# Autodesk Inventor assembly: 537245 FNC-12
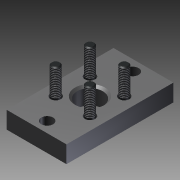
[picture p0: Inventor's stored thumbnail of the model, 180x180]
Saved by Autodesk Inventor 2011 SP1 (Build 150282100, 282)
## iProperties
Created: 2018-05-28
Part Number: 537245 FNC-12
Catalog Web Link: www.cadenas.de
Description: FNC-Flange mounting
Vendor: FESTO
Document SubType Name: Assembly
Designer: psAdmin
Manufacturer: FESTO
Mass: 79 g
Category: PARTsolutions
Company: FESTO
Title: 537245 FNC-12
Author: Cadenas PARTsolutions
Comments: Flange mounting
PSOL_IDENT_0: {$CADENAS_DATA\23d-libs\festo\parts\f\fnc\fnc_asmtab.prj},179 {VTYP=3D},{STYP=ASSTAB},{NB=537245 FNC
PSOL_IDENT_1: -12},{LINA=537245 FNC-12},{NN=FNC},{DATE=02.09.2015 15:05:29},{GEOMDATE=02.09.2015 15:05:29},{VERSIO
PSOL_IDENT_2: N=},{LINEID=80},{LINESUBID=-1},{WBVAR=}  {NB=537245 FNC-12},{LINA=537245 FNC-12},{KT=DUMMY},{TNR=537
PSOL_IDENT_3: 245},{TYP=FNC-12},{VERS=1},{D1=12.000},{D2=4.800},{D3=8.000},{E=28.000},{F=1.000},{FB=5.500},{MF=8.0
PSOL_IDENT_4: 00},{R=0.000},{T=3.000},{TF=40.000},{TG1=16.000},{UF=50.000},{CNSMASSEXACT=0.079},{ZZ=0},{DK=12},{D6
PSOL_IDENT_5: 912D=4.000},{D6912L=16.000},{PPATH=assemblies/fnc_asmtpl.prj}
NN: FNC
NT: Flange mounting
NB: 537245 FNC-12
NBSYN: $TNR. $TYP.
LINA: 537245 FNC-12
TNR: 537245
TYP: FNC-12
D1: 12.000
D2: 4.800
D3: 8.000
E: 28.000
F: 1.000
FB: 5.500
MF: 8.000
R: 0.000
T: 3.000
TF: 40.000
TG1: 16.000
UF: 50.000
CNSMASSEXACT: 0.079
SUPPLIER: FESTO
ARTICLENO: 537245 FNC-12
BOMINFO: 537245 FNC-12
CREATOR: CADENAS GmbH
## Documents named in this file (3)
- p:\temp\worker_3\2348_1500\cad_40_02018052900041801315782192d056f_000000_00_00_000001\537245 FNC-12.iam
- p:\temp\worker_3\2348_1500\cad_40_02018052900041801315782192d056f_000000_00_00_000001\537245 FNC-12---(F).ipt
- p:\temp\worker_3\2348_1500\cad_40_02018052900041801315782192d056f_000000_00_00_000001\DIN-6912 - M4x16(F).ipt
## Components (5 placed, 2 different names)
1. 537245 FNC-12---(F):1 — FNC_Schraube_1_XY@1 <-> MONTAGE_XY@2, FNC_Schraube_1_Z@1 <-> MONTAGE_Z@2, FNC_Schraube_2_XY@1 <-> MONTAGE_XY@3, FNC_Schraube_2_Z@1 <-> MONTAGE_Z@3, FNC_Schraube_2_YZ@1 <-> MONTAGE_YZ@3, FNC_Schraube_3_XY@1 <-> MONTAGE_XY@4, FNC_Schraube_3_Z@1 <-> MONTAGE_Z@4, FNC_Schraube_3_YZ@1 <-> MONTAGE_YZ@4, FNC_Schraube_4_XY@1 <-> MONTAGE_XY@5, FNC_Schraube_4_Z@1 <-> MONTAGE_Z@5
2. DIN-6912 - M4x16(F):1 — FNC_Schraube_1_XY@1 <-> MONTAGE_XY@2, FNC_Schraube_1_Z@1 <-> MONTAGE_Z@2
3. DIN-6912 - M4x16(F):2 — FNC_Schraube_2_XY@1 <-> MONTAGE_XY@3, FNC_Schraube_2_Z@1 <-> MONTAGE_Z@3, FNC_Schraube_2_YZ@1 <-> MONTAGE_YZ@3
4. DIN-6912 - M4x16(F):3 — FNC_Schraube_3_XY@1 <-> MONTAGE_XY@4, FNC_Schraube_3_Z@1 <-> MONTAGE_Z@4, FNC_Schraube_3_YZ@1 <-> MONTAGE_YZ@4
5. DIN-6912 - M4x16(F):4 — FNC_Schraube_4_XY@1 <-> MONTAGE_XY@5, FNC_Schraube_4_Z@1 <-> MONTAGE_Z@5
## Relationships (10: Flush 4, Mate 4, Angle 2)
- FNC_Schraube_1_XY@1 <-> MONTAGE_XY@2 [Flush]: 537245 FNC-12---(F):1 ↔ DIN-6912 - M4x16(F):1
- FNC_Schraube_1_Z@1 <-> MONTAGE_Z@2 [Mate]: 537245 FNC-12---(F):1 ↔ DIN-6912 - M4x16(F):1
- FNC_Schraube_2_XY@1 <-> MONTAGE_XY@3 [Flush]: 537245 FNC-12---(F):1 ↔ DIN-6912 - M4x16(F):2
- FNC_Schraube_2_Z@1 <-> MONTAGE_Z@3 [Mate]: 537245 FNC-12---(F):1 ↔ DIN-6912 - M4x16(F):2
- FNC_Schraube_2_YZ@1 <-> MONTAGE_YZ@3 [Angle] (0 deg): 537245 FNC-12---(F):1 ↔ DIN-6912 - M4x16(F):2
- FNC_Schraube_3_XY@1 <-> MONTAGE_XY@4 [Flush]: 537245 FNC-12---(F):1 ↔ DIN-6912 - M4x16(F):3
- FNC_Schraube_3_Z@1 <-> MONTAGE_Z@4 [Mate]: 537245 FNC-12---(F):1 ↔ DIN-6912 - M4x16(F):3
- FNC_Schraube_3_YZ@1 <-> MONTAGE_YZ@4 [Angle] (0 deg): 537245 FNC-12---(F):1 ↔ DIN-6912 - M4x16(F):3
- FNC_Schraube_4_XY@1 <-> MONTAGE_XY@5 [Flush]: 537245 FNC-12---(F):1 ↔ DIN-6912 - M4x16(F):4
- FNC_Schraube_4_Z@1 <-> MONTAGE_Z@5 [Mate]: 537245 FNC-12---(F):1 ↔ DIN-6912 - M4x16(F):4
